# Autodesk Inventor assembly: chwytak
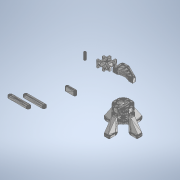
[picture p0: Inventor's stored thumbnail of the model, 180x180]
Saved by Autodesk Inventor 2022.3 (Build 263350000, 350)
## iProperties
Created: 2023-06-03
Part Number: chwytak
Document SubType Name: Assembly
Designer: komputer
Author: komputer
## Documents named in this file (11)
- C:\Users\komputer\Documents\Inventor\Warsztaty\chwytak.iam
- C:\Users\komputer\AppData\Local\Temp\Rar$DIa7596.38510\GripperBaseCircularUpper.ipt
- C:\Users\komputer\Documents\Inventor\Warsztaty\GripperBaseCircularLower.ipt
- C:\Users\komputer\AppData\Local\Temp\Rar$DIa7596.38510\Arm.ipt
- C:\Users\komputer\AppData\Local\Temp\Rar$DIa7596.38510\ArmMuscle.ipt
- C:\Users\komputer\AppData\Local\Temp\Rar$DIa7596.38510\ArmOuter.ipt
- C:\Users\komputer\AppData\Local\Temp\Rar$DIa7596.38510\CircularStandOff.ipt
- C:\Users\komputer\AppData\Local\Temp\Rar$DIa7596.38510\ClawShoulder.ipt
- C:\Users\komputer\AppData\Local\Temp\Rar$DIa7596.38510\GripperClaw.ipt
- C:\Users\komputer\AppData\Local\Temp\Rar$DIa7596.38510\GripperMotorHinges.ipt
- C:\Users\komputer\AppData\Local\Temp\Rar$DIa7596.38510\ShaftToScrewCoupler.ipt
## Components (16 placed, 10 different names)
1. Arm:1
2. ArmMuscle:1
3. ArmOuter:1
4. CircularStandOff:1 — Mate:13, Mate:14, Mate:21, Mate:23
5. ClawShoulder:1 — Mate:1, Mate:2, Mate:3
6. GripperBaseCircularLower:1 — Mate:21, Mate:22, Mate:23
7. GripperBaseCircularUpper:2 — Mate:1, Mate:2, Mate:3, Mate:4, Mate:5, Mate:6, Mate:7, Mate:8, Mate:9, Mate:10, Mate:11, Mate:12, Mate:13, Mate:14, Mate:15, Mate:16, Mate:17, Mate:18, Mate:19, Mate:20
8. GripperClaw:1
9. GripperMotorHinges:1
10. ShaftToScrewCoupler:1
11. ClawShoulder:2 — Mate:4, Mate:5, Mate:6
12. ClawShoulder:3 — Mate:7, Mate:8, Mate:9
13. ClawShoulder:4 — Mate:10, Mate:11, Mate:12
14. CircularStandOff:2 — Mate:15, Mate:18
15. CircularStandOff:3 — Mate:17, Mate:20
16. CircularStandOff:4 — Mate:16, Mate:19, Mate:22
## Relationships (23: Mate 23)
- Mate:1: ClawShoulder:1 ↔ GripperBaseCircularUpper:2
- Mate:2: ClawShoulder:1 ↔ GripperBaseCircularUpper:2
- Mate:3: ClawShoulder:1 ↔ GripperBaseCircularUpper:2
- Mate:4: GripperBaseCircularUpper:2 ↔ ClawShoulder:2
- Mate:5: GripperBaseCircularUpper:2 ↔ ClawShoulder:2
- Mate:6: GripperBaseCircularUpper:2 ↔ ClawShoulder:2
- Mate:7: GripperBaseCircularUpper:2 ↔ ClawShoulder:3
- Mate:8: GripperBaseCircularUpper:2 ↔ ClawShoulder:3
- Mate:9: GripperBaseCircularUpper:2 ↔ ClawShoulder:3
- Mate:10: GripperBaseCircularUpper:2 ↔ ClawShoulder:4
- Mate:11: GripperBaseCircularUpper:2 ↔ ClawShoulder:4
- Mate:12: GripperBaseCircularUpper:2 ↔ ClawShoulder:4
- Mate:13: CircularStandOff:1 ↔ GripperBaseCircularUpper:2
- Mate:14: CircularStandOff:1 ↔ GripperBaseCircularUpper:2
- Mate:15: GripperBaseCircularUpper:2 ↔ CircularStandOff:2
- Mate:16: GripperBaseCircularUpper:2 ↔ CircularStandOff:4
- Mate:17: GripperBaseCircularUpper:2 ↔ CircularStandOff:3
- Mate:18: GripperBaseCircularUpper:2 ↔ CircularStandOff:2
- Mate:19: GripperBaseCircularUpper:2 ↔ CircularStandOff:4
- Mate:20: GripperBaseCircularUpper:2 ↔ CircularStandOff:3
- Mate:21: CircularStandOff:1 ↔ GripperBaseCircularLower:1
- Mate:22: GripperBaseCircularLower:1 ↔ CircularStandOff:4
- Mate:23: CircularStandOff:1 ↔ GripperBaseCircularLower:1
